# Autodesk Inventor assembly: V-Belt transmission
Saved by Autodesk Inventor 2014 SP1 (Build 180222100, 222)
## iProperties
Created: 2013-11-09
Part Number: V-Belt transmission
Document SubType Name: Assembly
Designer: RyanHughes
ClientObjectVersion: 1
Author: RyanHughes
## Documents named in this file (2)
- C:\Users\Ryan\Desktop\sw\toss up 2ed A bot\drivetrain\one side of drive\Design Accelerator\V-Belt transmission1.iam
- C:\Users\Ryan\Desktop\sw\toss up 2ed A bot\drivetrain\one side of drive\Design Accelerator\V-Belt1.ipt
## Components (1 placed, 1 different names)
1. V-Belt:1
## Component patterns: (1 elements, first: V-Belt:1)
